# Autodesk Inventor assembly: Intake Full Assembly
(part 2 of 2)
- Mate:645: COTS_217-2592_VersaHub:3 ↔ COTS_91251A196_Black-Oxide Alloy Steel Socket Head Screw_5-8in:9
- Mate:646: COTS_91251A196_Black-Oxide Alloy Steel Socket Head Screw_5-8in:10 ↔ COTS_90631A009_8-32_Low-Strength Steel Nylon-Insert Locknut:11
- Mate:647: Intake Roller Plate:2 ↔ COTS_90631A009_8-32_Low-Strength Steel Nylon-Insert Locknut:11
- Mate:648: COTS_91251A196_Black-Oxide Alloy Steel Socket Head Screw_5-8in:8 ↔ COTS_90631A009_8-32_Low-Strength Steel Nylon-Insert Locknut:1
- Mate:649: Intake Roller Plate:2 ↔ COTS_90631A009_8-32_Low-Strength Steel Nylon-Insert Locknut:1
- Mate:650: COTS_91251A196_Black-Oxide Alloy Steel Socket Head Screw_5-8in:7 ↔ COTS_90631A009_8-32_Low-Strength Steel Nylon-Insert Locknut:12
- Mate:651: Intake Roller Plate:2 ↔ COTS_90631A009_8-32_Low-Strength Steel Nylon-Insert Locknut:12
- Mate:652: COTS_91251A196_Black-Oxide Alloy Steel Socket Head Screw_5-8in:12 ↔ COTS_90631A009_8-32_Low-Strength Steel Nylon-Insert Locknut:4
- Mate:653: Intake Roller Plate:2 ↔ COTS_90631A009_8-32_Low-Strength Steel Nylon-Insert Locknut:4
- Mate:654: COTS_91251A196_Black-Oxide Alloy Steel Socket Head Screw_5-8in:5 ↔ COTS_90631A009_8-32_Low-Strength Steel Nylon-Insert Locknut:8
- Mate:655: Intake Roller Plate:2 ↔ COTS_90631A009_8-32_Low-Strength Steel Nylon-Insert Locknut:8
- Mate:656: COTS_91251A196_Black-Oxide Alloy Steel Socket Head Screw_5-8in:9 ↔ COTS_90631A009_8-32_Low-Strength Steel Nylon-Insert Locknut:7
- Mate:657: Intake Roller Plate:2 ↔ COTS_90631A009_8-32_Low-Strength Steel Nylon-Insert Locknut:7
- Mate:658: COTS_91251A196_Black-Oxide Alloy Steel Socket Head Screw_5-8in:3 ↔ COTS_90631A009_8-32_Low-Strength Steel Nylon-Insert Locknut:5
- Mate:659: COTS_91251A196_Black-Oxide Alloy Steel Socket Head Screw_5-8in:2 ↔ COTS_90631A009_8-32_Low-Strength Steel Nylon-Insert Locknut:9
- Mate:660: COTS_91251A196_Black-Oxide Alloy Steel Socket Head Screw_5-8in:4 ↔ COTS_90631A009_8-32_Low-Strength Steel Nylon-Insert Locknut:10
- Mate:661: COTS_91251A196_Black-Oxide Alloy Steel Socket Head Screw_5-8in:6 ↔ COTS_90631A009_8-32_Low-Strength Steel Nylon-Insert Locknut:6
- Mate:662: COTS_91251A196_Black-Oxide Alloy Steel Socket Head Screw_5-8in:11 ↔ COTS_90631A009_8-32_Low-Strength Steel Nylon-Insert Locknut:2
- Mate:663: COTS_91251A196_Black-Oxide Alloy Steel Socket Head Screw_5-8in:1 ↔ COTS_90631A009_8-32_Low-Strength Steel Nylon-Insert Locknut:3
- Mate:664: Intake Roller Plate:1 ↔ COTS_90631A009_8-32_Low-Strength Steel Nylon-Insert Locknut:3
- Mate:665: Intake Roller Plate:1 ↔ COTS_90631A009_8-32_Low-Strength Steel Nylon-Insert Locknut:5
- Mate:666: Intake Roller Plate:1 ↔ COTS_90631A009_8-32_Low-Strength Steel Nylon-Insert Locknut:9
- Mate:667: Intake Roller Plate:1 ↔ COTS_90631A009_8-32_Low-Strength Steel Nylon-Insert Locknut:10
- Mate:668: Intake Roller Plate:1 ↔ COTS_90631A009_8-32_Low-Strength Steel Nylon-Insert Locknut:6
- Mate:669: Intake Roller Plate:1 ↔ COTS_90631A009_8-32_Low-Strength Steel Nylon-Insert Locknut:2
- Mate:670: Intake Roller Plate:1 ↔ COTS_92949A265_1-2in long Stainless Steel Button Head Screw:28
- Mate:674: Intake Roller Plate:1 ↔ COTS_92949A265_1-2in long Stainless Steel Button Head Screw:28
- Mate:675: COTS_WCP-0783_1.125ODHexBearing:19 ↔ INtk_010_Belt2:1
- Mate:676 (0.508 mm): COTS_WCP-0783_1.125ODHexBearing:14 ↔ INtk_010_Belt2:1
- Mate:677: COTS_HTD5M10mm15T_WCP-1420:4 ↔ INtk_010_Belt2:1
- Mate:678: COTS_WCP-0783_1.125ODHexBearing:14 ↔ INTK_009_Belt1:1
- Mate:679: INTK_006_Spacer6:1 ↔ INTK_009_Belt1:1
- Mate:680: COTW_HTD5M10mm12T_WCP-0076:1 ↔ INTK_009_Belt1:1
- Mate:681: COTS_WCP-0783_1.125ODHexBearing:20 ↔ INtk_010_Belt2:2
- Mate:682: COTS_WCP-0783_1.125ODHexBearing:15 ↔ INtk_010_Belt2:2
- Mate:683: COTS_HTD5M10mm15T_WCP-1420:1 ↔ INtk_010_Belt2:2
- Mate:684: COTS_WCP-0799_0.5inchHexShaftCollar:8 ↔ INTK_011_Belt3:1
- Mate:685: COTS_WCP-0799_0.5inchHexShaftCollar:7 ↔ INTK_011_Belt3:1
- Mate:687: COTS_WCP-0799_0.5inchHexShaftCollar:6 ↔ INTK_011_Belt3:2
- Mate:688: COTS_WCP-0799_0.5inchHexShaftCollar:5 ↔ INTK_011_Belt3:2
- Mate:690: COTS_WCP-0799_0.5inchHexShaftCollar:11 ↔ INTK_012_Belt4:1
- Mate:691: COTS_WCP-0799_0.5inchHexShaftCollar:9 ↔ INTK_012_Belt4:1
- Mate:692: COTS_HTD5M10mm18T_WCP-0563:4 ↔ INTK_012_Belt4:1
- Mate:693: COTS_WCP-0799_0.5inchHexShaftCollar:10 ↔ INTK_012_Belt4:2
- Mate:694: COTS_WCP-0799_0.5inchHexShaftCollar:12 ↔ INTK_012_Belt4:2
- Mate:695: Intake Roller Plate:2 ↔ INTK_012_Belt4:2
- Mate:696: INTK_005_Spacer5:6 ↔ INTK_013_Belt5:1
- Mate:697: INTK_005_Spacer5:7 ↔ INTK_013_Belt5:1
- Mate:698: COTS_HTD5M10mm18T_WCP-0563:15 ↔ INTK_013_Belt5:1
- Mate:699: INTK_005_Spacer5:4 ↔ INTK_013_Belt5:2
- Mate:700: INTK_005_Spacer5:2 ↔ INTK_013_Belt5:2
- Mate:701: COTS_HTD5M10mm18T_WCP-0563:11 ↔ INTK_013_Belt5:2
- Mate:702: INTK_005_Spacer5:3 ↔ INTK_014_Belt6:1
- Mate:703: COTS_WCP-0783_1.125ODHexBearing:17 ↔ INTK_014_Belt6:1
- Mate:704: COTS_HTD5M10mm18T_WCP-0563:1 ↔ INTK_014_Belt6:1
- Mate:705: Intake Roller Plate:1 ↔ COTS_92949A265_1-2in long Stainless Steel Button Head Screw:29
- Mate:706: Intake Roller Plate:1 ↔ COTS_92949A265_1-2in long Stainless Steel Button Head Screw:29
- Mate:707: COTS_REV-21-1650-V1.1:2 ↔ INTK_015_Spacer8:1
- Mate:708: COTS_REV-21-1650-V1.1:2 ↔ INTK_015_Spacer8:1
- Mate:709: COTS_WCP-0783_1.125ODHexBearing:19 ↔ INTK_005_Spacer5:5
- Mate:710: INTK_004_HexShaft6:1 ↔ INTK_005_Spacer5:4
- Mate:711: INTK_004_HexShaft6:2 ↔ INTK_005_Spacer5:2
- Mate:713: INTK_004_HexShaft6:3 ↔ INTK_005_Spacer5:1
- Mate:714: COTS_HTD5M10mm15T_WCP-1420:1 ↔ INtk_010_Belt2:2
- Mate:715: INTK_007_Spacer7:4 ↔ COTS_92949A265_1-2in long Stainless Steel Button Head Screw:7
- Mate:716: INTK_007_Spacer7:16 ↔ COTS_92949A265_1-2in long Stainless Steel Button Head Screw:16
- Mate:717: INTK_007_Spacer7:15 ↔ COTS_92949A265_1-2in long Stainless Steel Button Head Screw:15
- Mate:718: INTK_007_Spacer7:1 ↔ COTS_92949A265_1-2in long Stainless Steel Button Head Screw:18
- Mate:720: INTK_007_Spacer7:8 ↔ COTS_92949A265_1-2in long Stainless Steel Button Head Screw:24
- Mate:721: INTK_007_Spacer7:14 ↔ COTS_92949A265_1-2in long Stainless Steel Button Head Screw:14
- Mate:722: INTK_007_Spacer7:15 ↔ COTS_92949A265_1-2in long Stainless Steel Button Head Screw:15
- Mate:723: INTK_001_PulleyCover:1 ↔ INTK_006_Spacer6:1
- Mate:724: INTK_001_PulleyCover:1 ↔ COTS_WCP-0783_1.125ODHexBearing:19
- Mate:725: INTK_001_PulleyCover:1 ↔ COTS_WCP-0783_1.125ODHexBearing:19
- Mate:726: COTS_WCP-0783_1.125ODHexBearing:14 ↔ INTK_001_PulleyCover:1
- Mate:727: COTS_WCP-0783_1.125ODHexBearing:14 ↔ INTK_001_PulleyCover:1
- Mate:729: INTK_001_PulleyCover:1 ↔ COTS_WCP-0783_1.125ODHexBearing:22
- Mate:730: INTK_001_PulleyCover:1 ↔ COTS_WCP-0783_1.125ODHexBearing:21
- Mate:731: INTK_001_PulleyCover:1 ↔ COTS_WCP-0783_1.125ODHexBearing:22
- Mate:732: INTK_001_PulleyCover:1 ↔ INTK_007_Spacer7:14
- Mate:733: Intake Roller Plate:1 ↔ INTK_007_Spacer7:14
- Mate:734: INTK_001_PulleyCover:1 ↔ COTS_92949A265_1-2in long Stainless Steel Button Head Screw:14
- Mate:735: INTK_001_PulleyCover:1 ↔ INTK_007_Spacer7:15
- Mate:736: Intake Roller Plate:1 ↔ INTK_007_Spacer7:15
- Mate:737: INTK_001_PulleyCover:1 ↔ COTS_92949A265_1-2in long Stainless Steel Button Head Screw:15
- Mate:738: INTK_007_Spacer7:16 ↔ COTS_92949A265_1-2in long Stainless Steel Button Head Screw:19
- Mate:739: INTK_001_PulleyCover:1 ↔ INTK_007_Spacer7:16
- Mate:740: INTK_001_PulleyCover:1 ↔ COTS_92949A265_1-2in long Stainless Steel Button Head Screw:16
- Mate:741: INTK_007_Spacer7:4 ↔ COTS_92949A265_1-2in long Stainless Steel Button Head Screw:6
- Mate:742: INTK_001_PulleyCover:1 ↔ INTK_007_Spacer7:4
- Mate:743: INTK_001_PulleyCover:1 ↔ COTS_92949A265_1-2in long Stainless Steel Button Head Screw:7
- Mate:744: INTK_001_PulleyCover:1 ↔ COTS_92949A265_1-2in long Stainless Steel Button Head Screw:7
- Mate:745: INTK_007_Spacer7:8 ↔ COTS_92949A265_1-2in long Stainless Steel Button Head Screw:20
- Mate:746: INTK_001_PulleyCover:1 ↔ COTS_92949A265_1-2in long Stainless Steel Button Head Screw:24
- Mate:747: INTK_001_PulleyCover:1 ↔ INTK_007_Spacer7:1
- Mate:748: INTK_001_PulleyCover:1 ↔ COTS_92949A265_1-2in long Stainless Steel Button Head Screw:18
- Mate:749: Intake Roller Plate:1 ↔ COTS_92949A265_1-2in long Stainless Steel Button Head Screw:17
- Mate:750: INTK_001_PulleyCover:2 ↔ INTK_007_Spacer7:5
- Mate:751: INTK_001_PulleyCover:2 ↔ COTS_92949A265_1-2in long Stainless Steel Button Head Screw:5
- Mate:752: INTK_001_PulleyCover:2 ↔ COTS_92949A265_1-2in long Stainless Steel Button Head Screw:5
- Mate:753: INTK_001_PulleyCover:2 ↔ INTK_007_Spacer7:5
- Mate:754: INTK_001_PulleyCover:2 ↔ COTS_92949A265_1-2in long Stainless Steel Button Head Screw:3
- Mate:755: INTK_007_Spacer7:12 ↔ COTS_92949A265_1-2in long Stainless Steel Button Head Screw:3
- Mate:756: INTK_001_PulleyCover:2 ↔ INTK_007_Spacer7:12
- Mate:757: INTK_001_PulleyCover:2 ↔ COTS_92949A265_1-2in long Stainless Steel Button Head Screw:3
- Mate:758: INTK_001_PulleyCover:2 ↔ COTS_92949A265_1-2in long Stainless Steel Button Head Screw:2
- Mate:759: INTK_007_Spacer7:7 ↔ COTS_92949A265_1-2in long Stainless Steel Button Head Screw:2
- Mate:760: INTK_001_PulleyCover:2 ↔ COTS_92949A265_1-2in long Stainless Steel Button Head Screw:2
- Mate:761: INTK_001_PulleyCover:2 ↔ INTK_007_Spacer7:7
- Mate:762: INTK_001_PulleyCover:2 ↔ INTK_007_Spacer7:2
- Mate:763: INTK_001_PulleyCover:2 ↔ COTS_92949A265_1-2in long Stainless Steel Button Head Screw:4
- Mate:764: INTK_001_PulleyCover:2 ↔ COTS_92949A265_1-2in long Stainless Steel Button Head Screw:4
- Mate:765: INTK_001_PulleyCover:2 ↔ INTK_007_Spacer7:2
- Mate:766: INTK_001_PulleyCover:2 ↔ INTK_007_Spacer7:3
- Mate:767: INTK_001_PulleyCover:2 ↔ INTK_007_Spacer7:3
- Mate:768: INTK_007_Spacer7:3 ↔ COTS_92949A265_1-2in long Stainless Steel Button Head Screw:1
- Mate:769: INTK_001_PulleyCover:2 ↔ COTS_92949A265_1-2in long Stainless Steel Button Head Screw:1
- Mate:770: INTK_001_PulleyCover:2 ↔ INTK_007_Spacer7:11
- Mate:771: INTK_001_PulleyCover:2 ↔ INTK_007_Spacer7:11
- Mate:772: INTK_001_PulleyCover:2 ↔ COTS_92949A265_1-2in long Stainless Steel Button Head Screw:12
- Mate:773: INTK_001_PulleyCover:2 ↔ COTS_92949A265_1-2in long Stainless Steel Button Head Screw:12
- Mate:774: Intake Roller Plate:2 ↔ INTK_001_PulleyCover:2
- Mate:775: INTK_007_Spacer7:5 ↔ COTS_92949A265_1-2in long Stainless Steel Button Head Screw:27
- Mate:776: Intake Roller Plate:2 ↔ INTK_007_Spacer7:7
- Mate:777: COTS_WCP-0783_1.125ODHexBearing:15 ↔ INTK_001_PulleyCover:2
- Mate:778: INTK_001_PulleyCover:2 ↔ COTS_WCP-0783_1.125ODHexBearing:20
- Mate:779: INTK_001_PulleyCover:2 ↔ COTS_WCP-0783_1.125ODHexBearing:24
- Mate:780: INTK_001_PulleyCover:2 ↔ COTS_WCP-0783_1.125ODHexBearing:24
- Mate:781: INTK_001_PulleyCover:2 ↔ COTS_WCP-0783_1.125ODHexBearing:23
- Mate:782: Intake Roller Plate:2 ↔ COTS_92949A265_1-2in long Stainless Steel Button Head Screw:13
- Mate:783: Intake Roller Plate:2 ↔ COTS_92949A265_1-2in long Stainless Steel Button Head Screw:13
- Mate:784: COTS_HTD5M10mm18T_WCP-0563:5 ↔ INTK_011_Belt3:2
- Mate:785: COTS_HTD5M10mm18T_WCP-0563:16 ↔ INTK_011_Belt3:1
- Mate:786: Intake Roller Plate:1 ↔ COTS_92949A265_1-2in long Stainless Steel Button Head Screw:17
- Flush:32: INTK_004_HexShaft6:2 ↔ COTS_WCP-0783_1.125ODHexBearing:24
- Mate:787: INTK_001_PulleyCover:1 ↔ COTS_WCP-0783_1.125ODHexBearing:21
